# Autodesk Inventor assembly: ProtoModelMake
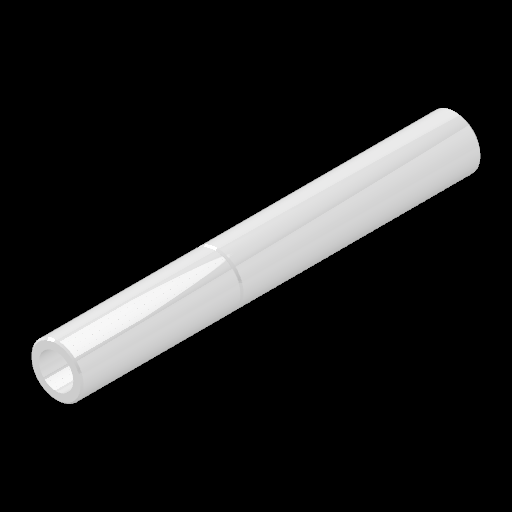
[picture p0: Inventor's stored thumbnail of the model, 512x512]
Saved by Autodesk Inventor 2023 (Build 270158000, 158)
## iProperties
Created: 2022-01-30
Part Number: ProtoModelMake
Document SubType Name: Assembly
Designer: Michael Lacey
Mass: 609.205 g
Surface Area: 774.58 cm^2
Volume: 225.632 cm^3
Density: 2.7 g/cm^3
Author: Michael Lacey
## Documents named in this file (3)
- C:\Users\foams\3D Objects\Light Saber\All Files Compiled\CAD\ProtoModelMake.iam
- C:\Users\foams\3D Objects\Light Saber\All Files Compiled\CAD\EndHilt.ipt
- C:\Users\foams\3D Objects\Light Saber\All Files Compiled\CAD\MainHilt.ipt
## Components (2 placed, 2 different names)
1. MainHilt:1 — Cylindrical:1, Mate:7
2. EndHilt:1 — Cylindrical:1, Mate:7
## Relationships (2: CylindricalJoint 1, Mate 1)
- Cylindrical:1: MainHilt:1 ↔ EndHilt:1
- Mate:7: MainHilt:1 ↔ EndHilt:1
